# Autodesk Inventor assembly: Assembly6
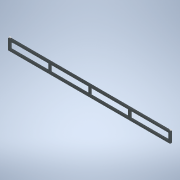
[picture p0: Inventor's stored thumbnail of the model, 180x180]
Saved by Autodesk Inventor 2021 (Build 250183000, 183)
## iProperties
Created: 2023-12-08
Part Number: Assembly6
Document SubType Name: Assembly
Designer: assman
Author: assman
## Documents named in this file (3)
- D:\3DPrinting\3DModels\roco\Assembly6.iam
- D:\3DPrinting\3DModels\roco\structure.ipt
- D:\3DPrinting\3DModels\roco\hinge_assembly.iam
## Components (3 placed, 2 different names)
1. structure:1 — Mate:1, Mate:2, Mate:3, Mate:4
2. hinge_assembly:1 [sub-assembly] — Mate:1, Mate:2
3. hinge_assembly:2 [sub-assembly] — Mate:3, Mate:4
## Relationships (4: Mate 4)
- Mate:1: structure:1 ↔ hinge_assembly:1
- Mate:2: structure:1 ↔ hinge_assembly:1
- Mate:3: structure:1 ↔ hinge_assembly:2
- Mate:4: structure:1 ↔ hinge_assembly:2
